# Autodesk Inventor assembly: Apparatus Master Assem V4.1
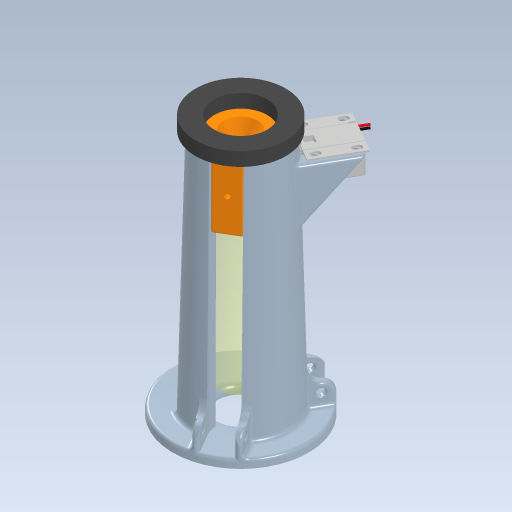
[picture p0: Inventor's stored thumbnail of the model, 512x512]
Saved by Autodesk Inventor 2023 (Build 270158000, 158)
## iProperties
Created: 2022-10-01
Part Number: Apparatus Master Assem V4.1
Document SubType Name: Assembly
Designer: david
Author: david
## Documents named in this file (7)
- C:\Users\Dave\Documents\GrabCAD\Chalk Bot\Chalkbot1.0\Apparatus\V4\Apparatus Master Assem V4.1.iam
- C:\Users\Dave\Documents\GrabCAD\Chalk Bot\Chalkbot1.0\Apparatus\V4\Tower pt2.ipt
- C:\Users\Dave\Documents\GrabCAD\Chalk Bot\Chalkbot1.0\Apparatus\V4\Slider V9 (2mm pitch).ipt
- C:\Users\Dave\Documents\GrabCAD\Chalk Bot\Chalkbot1.0\Apparatus\V4\Cap for Tower pt2.ipt
- C:\Users\Dave\Documents\GrabCAD\Chalk Bot\Chalkbot1.0\Apparatus\V3\Purchased Parts\Solenoid Lock.ipt
- C:\Users\Dave\Documents\GrabCAD\Chalk Bot\Chalkbot1.0\Apparatus\V3\Purchased Parts\Chalk.ipt
- C:\Users\Dave\Documents\GrabCAD\Chalk Bot\Chalkbot1.0\Apparatus\V3\Chalk Holder\Collet Ring V5.2 (2mm p).ipt
## Components (6 placed, 6 different names)
1. Tower pt2:1 — Insert:1, Cylindrical:1, Rigid:1
2. Slider V8 (4mm pitch):1 — Cylindrical:1, Mate:1, Insert:2
3. Cap for Tower pt2:1 — Insert:1
4. Solenoid Lock:1 — Rigid:1
5. Chalk:1 — Mate:1
6. Collet Ring V5.2 (2mm p):1 — Insert:2
## Relationships (5: Insert 2, CylindricalJoint 1, WeldJoint 1, Mate 1)
- Insert:1: Tower pt2:1 ↔ Cap for Tower pt2:1
- Cylindrical:1: Tower pt2:1 ↔ Slider V8 (4mm pitch):1
- Rigid:1 [WeldJoint]: Tower pt2:1 ↔ Solenoid Lock:1
- Mate:1: Slider V8 (4mm pitch):1 ↔ Chalk:1
- Insert:2 (-8 mm): Slider V8 (4mm pitch):1 ↔ Collet Ring V5.2 (2mm p):1
